# Autodesk Inventor assembly: Macrolight
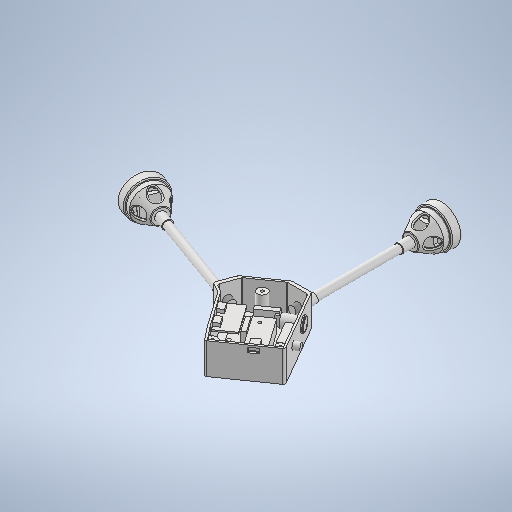
[picture p0: Inventor's stored thumbnail of the model, 512x512]
Saved by Autodesk Inventor 2025.1 (Build 291241000, 241)
## iProperties
Created: 2025-01-26
Part Number: Macrolight
Document SubType Name: Assembly
Designer: joebe
Author: joebe
## Documents named in this file (12)
- C:\Users\joebe\OneDrive\Documents\Projekte\Macrolampe\CAD\Baugruppen\Macrolight.iam
- C:\Users\joebe\OneDrive\Documents\Projekte\Macrolampe\CAD\Einzelteile\Kühler.ipt
- C:\Users\joebe\OneDrive\Documents\Projekte\Macrolampe\CAD\Einzelteile\LampenFront.ipt
- C:\Users\joebe\OneDrive\Documents\Projekte\Macrolampe\CAD\Einzelteile\LED-Schirm.ipt
- C:\Users\joebe\OneDrive\Documents\Projekte\Macrolampe\CAD\Einzelteile\Schwarnenhals.ipt
- C:\Users\joebe\OneDrive\Documents\Projekte\Macrolampe\CAD\Einzelteile\Deckel.ipt
- C:\Users\joebe\OneDrive\Documents\Projekte\Macrolampe\CAD\Einzelteile\Gehaueseunterteil.ipt
- C:\Users\joebe\OneDrive\Documents\Projekte\Macrolampe\CAD\Einzelteile\Platine.ipt
- C:\Users\joebe\OneDrive\Documents\Projekte\Macrolampe\CAD\Einzelteile\Knopf.ipt
- C:\Users\joebe\OneDrive\Documents\Projekte\Macrolampe\CAD\Einzelteile\encoder.ipt
- C:\Users\joebe\OneDrive\Documents\Projekte\Macrolampe\CAD\Einzelteile\hotshouh mount.ipt
- C:\Users\joebe\OneDrive\Documents\Projekte\Macrolampe\CAD\Einzelteile\Deckel_oberteil.ipt
## Components (16 placed, 11 different names)
1. Gehaueseunterteil:1 — Passend:13, Passend:14, Passend:15, Passend:16, Passend:17, Winkel:1, Winkel:2, Passend:26, Passend:27, Passend:28, Passend:29, Passend:30, Passend:31, Passend:32, Fluchtend:1, Fluchtend:2, Fluchtend:3, Fluchtend:4
2. Platine:1 — Passend:13, Passend:30, Passend:31
3. Knopf:1 — Passend:14, Passend:17, Winkel:2
4. encoder:1 — Passend:15, Passend:16, Winkel:1
5. Kühler:2
6. LampenFront:2
7. LED-Schirm:2
8. Schwarnenhals:2 — Passend:26, Passend:27
9. Deckel:2
10. Kühler:3 — Passend:35
11. LampenFront:3 — Passend:33, Passend:34, Passend:35, Passend:36, Passend:37, Passend:38
12. LED-Schirm:3 — Passend:36, Passend:39
13. Deckel:3 — Passend:34, Passend:38, Passend:39
14. Schwarnenhals:3 — Passend:28, Passend:29, Passend:33, Passend:37
15. hotshouh mount:2 — Passend:32, Fluchtend:1, Fluchtend:2
16. Deckel_oberteil:1 — Fluchtend:3, Fluchtend:4
## Relationships (33: Mate 27, Flush 4, Angle 2)
- Passend:13 [Mate] (0.5 mm): Gehaueseunterteil:1 ↔ Platine:1
- Passend:14 [Mate]: Gehaueseunterteil:1 ↔ Knopf:1
- Passend:15 [Mate]: Gehaueseunterteil:1 ↔ encoder:1
- Passend:16 [Mate]: Gehaueseunterteil:1 ↔ encoder:1
- Passend:17 [Mate]: Gehaueseunterteil:1 ↔ Knopf:1
- Winkel:1 [Angle] (0 deg): Gehaueseunterteil:1 ↔ encoder:1
- Winkel:2 [Angle] (0 deg): Gehaueseunterteil:1 ↔ Knopf:1
- [Mate]: LampenFront:2 ↔ Schwarnenhals:2
- [Mate]: LampenFront:2 ↔ Schwarnenhals:2
- [Mate]: Kühler:2 ↔ LampenFront:2
- [Mate]: Kühler:2 ↔ LampenFront:2
- [Mate]: Kühler:2 ↔ LED-Schirm:2
- [Mate]: LampenFront:2 ↔ LED-Schirm:2
- [Mate]: LampenFront:2 ↔ Deckel:2
- [Mate]: LED-Schirm:2 ↔ Deckel:2
- Passend:26 [Mate]: Gehaueseunterteil:1 ↔ Schwarnenhals:2
- Passend:27 [Mate]: Gehaueseunterteil:1 ↔ Schwarnenhals:2
- Passend:28 [Mate]: Gehaueseunterteil:1 ↔ Schwarnenhals:3
- Passend:29 [Mate]: Gehaueseunterteil:1 ↔ Schwarnenhals:3
- Passend:30 [Mate] (8 mm): Gehaueseunterteil:1 ↔ Platine:1
- Passend:31 [Mate]: Gehaueseunterteil:1 ↔ Platine:1
- Passend:32 [Mate]: Gehaueseunterteil:1 ↔ hotshouh mount:2
- Fluchtend:1 [Flush] (20 mm): Gehaueseunterteil:1 ↔ hotshouh mount:2
- Fluchtend:2 [Flush]: Gehaueseunterteil:1 ↔ hotshouh mount:2
- Fluchtend:3 [Flush]: Gehaueseunterteil:1 ↔ Deckel_oberteil:1
- Fluchtend:4 [Flush]: Gehaueseunterteil:1 ↔ Deckel_oberteil:1
- Passend:33 [Mate]: LampenFront:3 ↔ Schwarnenhals:3
- Passend:34 [Mate]: LampenFront:3 ↔ Deckel:3
- Passend:35 [Mate]: Kühler:3 ↔ LampenFront:3
- Passend:36 [Mate]: LampenFront:3 ↔ LED-Schirm:3
- Passend:37 [Mate]: LampenFront:3 ↔ Schwarnenhals:3
- Passend:38 [Mate]: LampenFront:3 ↔ Deckel:3
- Passend:39 [Mate]: LED-Schirm:3 ↔ Deckel:3
## Named parameters: d19_d7 = 0 mm, d20_d8 = 0 mm, d21_d0 = 0 mm, d22_d1 = 0 mm, d23_d2 = 0 mm, d24_d3 = 0 mm, d25_d5 = 0 mm, d26_d6 = 0 mm
